# Autodesk Inventor assembly: shoulder2_elbow_strain_sensor_away
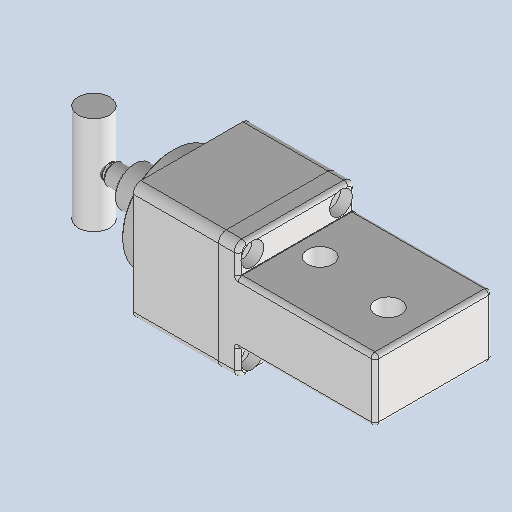
[picture p0: Inventor's stored thumbnail of the model, 512x512]
Saved by Autodesk Inventor 2024 (Build 280153000, 153)
## iProperties
Created: 2025-08-07
Part Number: shoulder2_elbow_strain_sensor_away
Document SubType Name: Assembly
Designer: HosodaLab2
Author: HosodaLab2
## Documents named in this file (6)
- C:\Users\HosodaLab2\OneDrive - Kyoto University\ドキュメント\Inventor\arm\shoulder2_elbow_strain_sensor_away.iam
- C:\Users\HosodaLab2\OneDrive - Kyoto University\ドキュメント\Inventor\arm\NewPart2.ipt
- C:\Users\HosodaLab2\OneDrive - Kyoto University\ドキュメント\Inventor\arm\C-LHFR5.ipt
- C:\Users\HosodaLab2\OneDrive - Kyoto University\ドキュメント\Inventor\arm\NewPart1.ipt
- C:\Users\HosodaLab2\OneDrive - Kyoto University\ドキュメント\Inventor\arm\SCLBRU5-35_0_D.ipt
- C:\Users\HosodaLab2\OneDrive - Kyoto University\ドキュメント\Inventor\arm\strain_sensor_jig.ipt
## Components (5 placed, 5 different names)
1. NewPart2:1 — 回転:1, 回転:2
2. C-LHFR5:1 — 回転:4, 回転:5
3. NewPart1:1 — 回転:1, 回転:2, 回転:3, 回転:4, 回転:5
4. SCLBRU5-35_0_D:1 — 回転:3, 回転:6
5. strain_sensor_jig:1 — 回転:6
## Relationships (6: RevoluteJoint 6)
- 回転:1 [RevoluteJoint]: NewPart2:1 ↔ NewPart1:1
- 回転:2 [RevoluteJoint]: NewPart2:1 ↔ NewPart1:1
- 回転:3 [RevoluteJoint]: NewPart1:1 ↔ SCLBRU5-35_0_D:1
- 回転:4 [RevoluteJoint]: C-LHFR5:1 ↔ NewPart1:1
- 回転:5 [RevoluteJoint]: C-LHFR5:1 ↔ NewPart1:1
- 回転:6 [RevoluteJoint]: SCLBRU5-35_0_D:1 ↔ strain_sensor_jig:1
